# Autodesk Inventor assembly: Plate_Ass
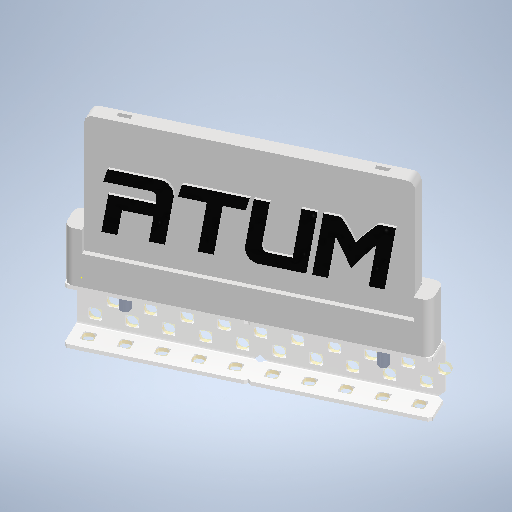
[picture p0: Inventor's stored thumbnail of the model, 512x512]
Saved by Autodesk Inventor 2025.2 (Build 292293000, 293)
## iProperties
Created: 2024-12-05
Part Number: Plate_Ass
Document SubType Name: Assembly
Designer: AtuStem
Author: AtuStem
## Documents named in this file (6)
- C:\Users\hmath\OneDrive\Documents\GitHub\ATUM-V5RC-High-Stakes-CAD\Plate_Ass.iam
- C:\Users\hmath\OneDrive\Documents\GitHub\ATUM-V5RC-High-Stakes-CAD\Protobot\Hunter Mathis\plate holder.ipt
- C:\Users\hmath\OneDrive\Documents\GitHub\ATUM-V5RC-High-Stakes-CAD\Protobot\Hunter Mathis\custom plate.ipt
- C:\Users\hmath\OneDrive\Documents\GitHub\ATUM-V5RC-High-Stakes-CAD\VEX-CAD-Inventor\Structure\C Channel\Aluminum 1x2x1\Alu C 1x2x1x10.ipt
- C:\Users\hmath\OneDrive\Documents\GitHub\ATUM-V5RC-High-Stakes-CAD\VEX-CAD-Inventor\Structure\Hardware\Screw Steel - Star\SScrew Star Smooth .500.ipt
- C:\Users\AtuStem\Documents\GitHub\ATUM-V5RC-High-Stakes-CAD\VEX-CAD-Inventor\Structure\Hardware\Screw Steel - Star.ipt
## Components (5 placed, 4 different names)
1. plate holder:3 — Mate:1, Mate:8, Mate:9, Mate:11, Mate:12, Mate:13
2. custom plate:1 — Mate:11, Mate:12, Mate:13
3. Alu C 1x2x1x10:1 — Mate:1, Mate:3, Mate:4, Mate:8, Mate:9
4. SScrew Star Smooth .500:1 — Mate:4
5. SScrew Star Smooth .500:2 — Mate:3
## Relationships (8: Mate 8)
- Mate:1: plate holder:3 ↔ Alu C 1x2x1x10:1
- Mate:3: Alu C 1x2x1x10:1 ↔ SScrew Star Smooth .500:2
- Mate:4: Alu C 1x2x1x10:1 ↔ SScrew Star Smooth .500:1
- Mate:8: plate holder:3 ↔ Alu C 1x2x1x10:1
- Mate:9: plate holder:3 ↔ Alu C 1x2x1x10:1
- Mate:11: plate holder:3 ↔ custom plate:1
- Mate:12: plate holder:3 ↔ custom plate:1
- Mate:13: plate holder:3 ↔ custom plate:1
